# Autodesk Inventor assembly: Assembly1
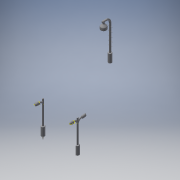
[picture p0: Inventor's stored thumbnail of the model, 180x180]
Saved by Autodesk Inventor 2018 (Build 220112000, 112)
## iProperties
Created: 2018-12-13
Part Number: Assembly1
Document SubType Name: Assembly
Designer: petal
Author: petal
## Documents named in this file (9)
- D:\OneDrive\3D modely\lampa\inventor_files\lampa.iam
- D:\OneDrive\3D modely\lampa\inventor_files\lampa.ipt
- D:\OneDrive\3D modely\lampa\inventor_files\3,5mm jack.ipt
- D:\OneDrive\3D modely\lampa\inventor_files\ledka.ipt
- D:\OneDrive\3D modely\lampa\inventor_files\lampa_MIR.ipt
- D:\OneDrive\3D modely\lampa\inventor_files\lampa_dual.ipt
- D:\OneDrive\3D modely\lampa\inventor_files\lampa_dual_MIR.ipt
- D:\OneDrive\3D modely\lampa\inventor_files\lampa_nadrazni.ipt
- D:\OneDrive\3D modely\lampa\inventor_files\lampa_nadrazni_MIR.ipt
## Components (8 placed, 8 different names)
1. lampa:1 — Mate:1, Mate:2, Mate:3
2. 3,5mm jack:1 — Mate:1
3. ledka:1 — Mate:2, Mate:3
4. lampa_MIR:1
5. lampa_dual:1
6. lampa_dual_MIR:1
7. lampa_nadrazni:1
8. lampa_nadrazni_MIR:1
## Relationships (3: Mate 3)
- Mate:1: lampa:1 ↔ 3,5mm jack:1
- Mate:2: lampa:1 ↔ ledka:1
- Mate:3: lampa:1 ↔ ledka:1
